# Autodesk Inventor assembly: Zespół1
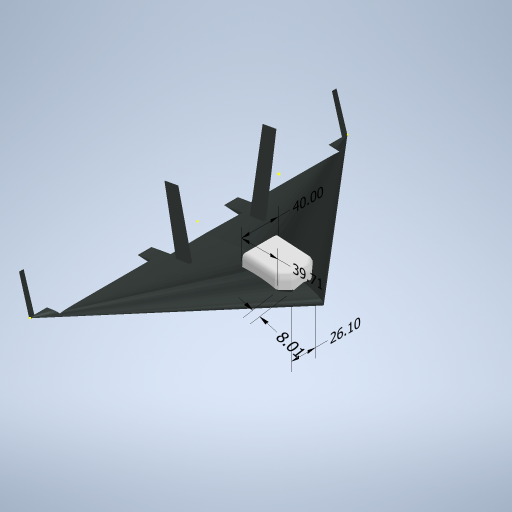
[picture p0: Inventor's stored thumbnail of the model, 512x512]
Saved by Autodesk Inventor 2023 (Build 270158000, 158)
## iProperties
Created: 2024-02-07
Part Number: Zespół1
Document SubType Name: Assembly
Designer: domin
Author: domin
## Documents named in this file (4)
- C:\Users\domin\projekty\OPIUM\fuselage\Zespół1.iam
- C:\Users\domin\projekty\OPIUM\fuselage\airfoil_MIR2.ipt
- C:\Users\domin\projekty\OPIUM\fuselage\airfoil_MIR1_MIR.ipt
- C:\Users\domin\projekty\OPIUM\fuselage\Część1.ipt
## Components (3 placed, 3 different names)
1. airfoil_MIR2:1 — Symetria:2
2. airfoil_MIR1_MIR:1 — Symetria:2, Zestawiające:1
3. Część1:1 — Zestawiające:1
## Relationships (2: Symmetry 1, Mate 1)
- Symetria:2 [Symmetry]: airfoil_MIR2:1 ↔ airfoil_MIR1_MIR:1
- Zestawiające:1 [Mate]: airfoil_MIR1_MIR:1 ↔ Część1:1
